# Autodesk Inventor assembly: derive_base_plate_bottom_v6
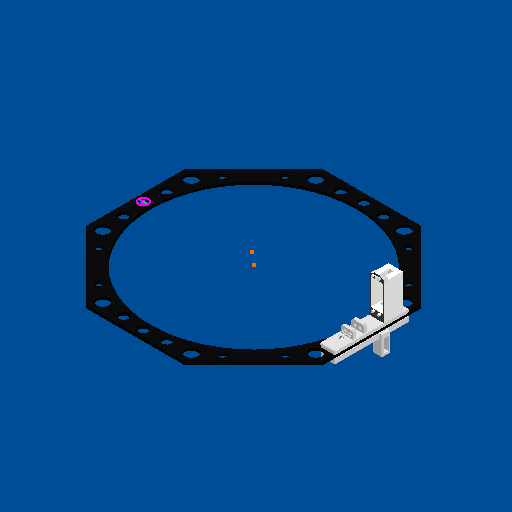
[picture p0: Inventor's stored thumbnail of the model, 512x512]
Saved by Autodesk Inventor 2026.2 (Build 302298000, 298)
## iProperties
Created: 2026-02-19
Part Number: derive_base_plate_bottom_v6
Document SubType Name: Assembly
Designer: Thoma
Author: Thoma
## Documents named in this file (9)
- C:\Users\Thoma\OneDrive\Desktop\dir\telescope_cover\cover\derive_base_plate_bottom_v6.iam
- C:\Users\Thoma\OneDrive\Desktop\dir\telescope_cover\cover\base_plate_bottom_v6.ipt
- C:\Users\Thoma\OneDrive\Desktop\dir\telescope_cover\telescope\version_4\Telescope_End.ipt
- C:\Users\Thoma\OneDrive\Desktop\dir\telescope_cover\cover\Base_plate_v15.ipt
- C:\Users\Thoma\OneDrive\Documents\Inventor\Content Center Files\R2026\en-US\ISO 7092\ISO 7092 - ST 4 - 140 HV.ipt
- C:\Users\Thoma\OneDrive\Documents\Inventor\Content Center Files\R2026\en-US\ISO 4762(2)\ISO 4762 - M4 x 20ISO.ipt
- C:\Users\Thoma\OneDrive\Documents\Inventor\Content Center Files\R2026\en-US\ISO 4032(2)\ISO 4032 - M4 - ISO.ipt
- C:\Users\Thoma\OneDrive\Documents\Inventor\Content Center Files\R2026\en-US\ISO 4762(2)\ISO 4762 - M4 x 30ISO.ipt
- C:\Users\Thoma\OneDrive\Documents\Inventor\Content Center Files\R2026\en-US\ISO 7093 A\ISO 7093 A - ST 4 - 140 HV .ipt
## Components (11 placed, 8 different names)
1. base_plate_bottom_v6:1 — Mate:4, Flush:1, Flush:2, Mate:5, Mate:7, Mate:8, Mate:9, Mate:11, Mate:12
2. Telescope_End:1 — Mate:1, Mate:2, Mate:3, Mate:4
3. Base_plate_v15:1 — Mate:1, Mate:2, Mate:3, Flush:1, Flush:2, Mate:6, Mate:10
4. ISO 7092 ST 4 - 140 HV:1 — Mate:5, Mate:6, Insert:1
5. ISO 4762 M4 x 20:1 — Insert:1
6. ISO 7092 ST 4 - 140 HV:2 — Mate:7, Mate:8, Insert:2
7. ISO 4032 M4:1 — Insert:2
8. ISO 7092 ST 4 - 140 HV:3 — Mate:9, Mate:10, Insert:3
9. ISO 4762 M4 x 30:1 — Insert:3
10. ISO 7093 A ST 4 - 140 HV - A:1 — Mate:11, Mate:12, Insert:4
11. ISO 4032 M4:2 — Insert:4
## Relationships (18: Mate 12, Insert 4, Flush 2)
- Mate:1: Telescope_End:1 ↔ Base_plate_v15:1
- Mate:2: Telescope_End:1 ↔ Base_plate_v15:1
- Mate:3: Telescope_End:1 ↔ Base_plate_v15:1
- Mate:4: base_plate_bottom_v6:1 ↔ Telescope_End:1
- Flush:1: base_plate_bottom_v6:1 ↔ Base_plate_v15:1
- Flush:2: base_plate_bottom_v6:1 ↔ Base_plate_v15:1
- Mate:5: base_plate_bottom_v6:1 ↔ ISO 7092 ST 4 - 140 HV:1
- Mate:6: Base_plate_v15:1 ↔ ISO 7092 ST 4 - 140 HV:1
- Insert:1: ISO 7092 ST 4 - 140 HV:1 ↔ ISO 4762 M4 x 20:1
- Mate:7: base_plate_bottom_v6:1 ↔ ISO 7092 ST 4 - 140 HV:2
- Mate:8: base_plate_bottom_v6:1 ↔ ISO 7092 ST 4 - 140 HV:2
- Insert:2: ISO 7092 ST 4 - 140 HV:2 ↔ ISO 4032 M4:1
- Mate:9: base_plate_bottom_v6:1 ↔ ISO 7092 ST 4 - 140 HV:3
- Mate:10: Base_plate_v15:1 ↔ ISO 7092 ST 4 - 140 HV:3
- Insert:3: ISO 7092 ST 4 - 140 HV:3 ↔ ISO 4762 M4 x 30:1
- Mate:11: base_plate_bottom_v6:1 ↔ ISO 7093 A ST 4 - 140 HV - A:1
- Mate:12: base_plate_bottom_v6:1 ↔ ISO 7093 A ST 4 - 140 HV - A:1
- Insert:4: ISO 7093 A ST 4 - 140 HV - A:1 ↔ ISO 4032 M4:2
